# Autodesk Inventor assembly: Robot
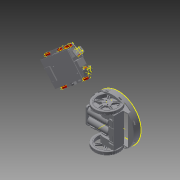
[picture p0: Inventor's stored thumbnail of the model, 180x180]
Saved by Autodesk Inventor 2014 (Build 180170000, 170)
## iProperties
Created: 2013-06-25
Part Number: Robot
Document SubType Name: Assembly
Designer: Felix
Author: Felix
## Documents named in this file (9)
- C:\Users\hanse\Desktop\Beep\Hardware\3D-CAD\Robot.iam
- C:\Users\hanse\Desktop\Beep\Hardware\3D-CAD\parts\Pololu_gear_motor_1_180\gear_motor.iam
- C:\Users\hanse\Desktop\Beep\Hardware\3D-CAD\parts\Pololu_Wheel_6mm\Wheel.iam
- C:\Users\hanse\Desktop\Beep\Hardware\3D-CAD\parts\battery_holder\holder_with_batteries_18500.iam
- C:\Users\hanse\Desktop\Beep\Hardware\3D-CAD\parts\battery_holder\holder_with_batteries_18650.iam
- C:\Users\Felix\Documents\Inventor\Content Center Files\R2014\de-DE\ISO 7046-1(1)\ISO 7046-1 - M2 x 8 - 4.8 - HDIN EN ISO.ipt
- C:\Users\hanse\Desktop\Beep\Hardware\3D-CAD\case\base.ipt
- C:\Users\hanse\Desktop\Beep\Hardware\3D-CAD\parts\electronic\BEEP\components\HSDL-9100-024\HSDL-9100.iam
- C:\Users\hanse\Desktop\Beep\Hardware\3D-CAD\parts\electronic\pcb_assembly.iam
## Components (18 placed, 8 different names)
1. gear_motor:1 [sub-assembly] — Passend:1, Passend:5, Passend:6, Passend:7, Fluchtend:3, Passend:13, Passend:14, Passend:16, Passend:18, Passend:19, Passend:24
2. gear_motor:2 [sub-assembly] — Passend:1, Passend:2, Passend:3, Passend:4, Fluchtend:3, Fluchtend:4, Fluchtend:5, Passend:12, Passend:15
3. Wheel:1 [sub-assembly] — Passend:5, Passend:6, Passend:7, Passend:24
4. Wheel:2 [sub-assembly] — Passend:2, Passend:3, Passend:4
5. holder_with_batteries_18500:1 [sub-assembly] — Fluchtend:4, Passend:13, Passend:14, Passend:15, Fluchtend:6
6. holder_with_batteries_18650:1 [sub-assembly] — Fluchtend:5, Passend:12, Passend:16, Passend:20, Passend:21, Passend:22, Passend:23
7. DIN EN ISO 7046-1 H M2 x 8 - 4.8 - H:1 — Passend:20, Passend:23
8. DIN EN ISO 7046-1 H M2 x 8 - 4.8 - H:2 — Passend:21, Passend:22
9. HSDL-9100:4 [sub-assembly] — Fluchtend:35
10. base:1 — Fluchtend:6, Passend:26, Passend:27, Fluchtend:11, Fluchtend:31, Fluchtend:12, Fluchtend:13, Fluchtend:32, Fluchtend:33, Fluchtend:34, Fluchtend:35
11. HSDL-9100:1 [sub-assembly] — Fluchtend:33
12. HSDL-9100:2 [sub-assembly] — Fluchtend:32
13. HSDL-9100:3 [sub-assembly] — Fluchtend:34
14. HSDL-9100:5 [sub-assembly] — Fluchtend:31
15. HSDL-9100:6 [sub-assembly] — Fluchtend:11
16. HSDL-9100:7 [sub-assembly] — Fluchtend:13
17. HSDL-9100:8 [sub-assembly] — Fluchtend:12
18. pcb_assembly:1 [sub-assembly]
## Relationships (34: Mate 22, Flush 12)
- Passend:1 [Mate]: gear_motor:1 ↔ gear_motor:2
- Passend:2 [Mate]: gear_motor:2 ↔ Wheel:2
- Passend:3 [Mate]: gear_motor:2 ↔ Wheel:2
- Passend:4 [Mate]: gear_motor:2 ↔ Wheel:2
- Passend:5 [Mate]: gear_motor:1 ↔ Wheel:1
- Passend:6 [Mate]: gear_motor:1 ↔ Wheel:1
- Passend:7 [Mate]: gear_motor:1 ↔ Wheel:1
- Fluchtend:3 [Flush]: gear_motor:1 ↔ gear_motor:2
- Fluchtend:4 [Flush]: gear_motor:2 ↔ holder_with_batteries_18500:1
- Fluchtend:5 [Flush]: gear_motor:2 ↔ holder_with_batteries_18650:1
- Passend:12 [Mate]: gear_motor:2 ↔ holder_with_batteries_18650:1
- Passend:13 [Mate]: gear_motor:1 ↔ holder_with_batteries_18500:1
- Passend:14 [Mate]: gear_motor:1 ↔ holder_with_batteries_18500:1
- Passend:15 [Mate]: gear_motor:2 ↔ holder_with_batteries_18500:1
- Passend:16 [Mate]: gear_motor:1 ↔ holder_with_batteries_18650:1
- Passend:18 [Mate]: gear_motor:1
- Passend:19 [Mate]: gear_motor:1
- Passend:20 [Mate]: holder_with_batteries_18650:1 ↔ DIN EN ISO 7046-1 H M2 x 8 - 4.8 - H:1
- Passend:21 [Mate]: holder_with_batteries_18650:1 ↔ DIN EN ISO 7046-1 H M2 x 8 - 4.8 - H:2
- Passend:22 [Mate]: holder_with_batteries_18650:1 ↔ DIN EN ISO 7046-1 H M2 x 8 - 4.8 - H:2
- Passend:23 [Mate]: holder_with_batteries_18650:1 ↔ DIN EN ISO 7046-1 H M2 x 8 - 4.8 - H:1
- Passend:24 [Mate]: gear_motor:1 ↔ Wheel:1
- Fluchtend:6 [Flush]: holder_with_batteries_18500:1 ↔ base:1
- Passend:26 [Mate]: base:1
- Passend:27 [Mate]: base:1
- Passend:28 [Mate]
- Fluchtend:11 [Flush]: base:1 ↔ HSDL-9100:6
- Fluchtend:31 [Flush]: base:1 ↔ HSDL-9100:5
- Fluchtend:12 [Flush]: base:1 ↔ HSDL-9100:8
- Fluchtend:13 [Flush]: base:1 ↔ HSDL-9100:7
- Fluchtend:32 [Flush]: base:1 ↔ HSDL-9100:2
- Fluchtend:33 [Flush]: base:1 ↔ HSDL-9100:1
- Fluchtend:34 [Flush]: base:1 ↔ HSDL-9100:3
- Fluchtend:35 [Flush]: HSDL-9100:4 ↔ base:1
